# Autodesk Inventor assembly: TheLightWithinYou-ManualAttachment
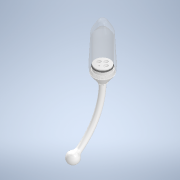
[picture p0: Inventor's stored thumbnail of the model, 180x180]
Saved by Autodesk Inventor 2021 (Build 250183000, 183)
## iProperties
Created: 2021-08-13
Part Number: TheLightWithinYou-ManualAttachment
Document SubType Name: Assembly
Designer: incep
Author: incep
## Documents named in this file (4)
- C:\Users\incep\Desktop\3D Printer Stuff\TheLightWithinYou\TheLightWithinYou-ManualAttachment.iam
- C:\Users\incep\Desktop\3D Printer Stuff\TheLightWithinYou\Bottom-V3-handle.ipt
- C:\Users\incep\Desktop\3D Printer Stuff\TheLightWithinYou\R-22-O-ring.ipt
- C:\Users\incep\Desktop\3D Printer Stuff\TheLightWithinYou\Upper-Threaded-v2.ipt
## Components (3 placed, 3 different names)
1. Bottom-V3-handle:1 — Mate:1, Flush:1, Mate:2, Mate:3
2. R-22-O-ring:1 — Mate:1, Flush:1
3. Upper-Threaded-v2:1 — Mate:2, Mate:3, Mate:4
## Relationships (5: Mate 4, Flush 1)
- Mate:1: Bottom-V3-handle:1 ↔ R-22-O-ring:1
- Flush:1: Bottom-V3-handle:1 ↔ R-22-O-ring:1
- Mate:2: Bottom-V3-handle:1 ↔ Upper-Threaded-v2:1
- Mate:3: Bottom-V3-handle:1 ↔ Upper-Threaded-v2:1
- Mate:4: Upper-Threaded-v2:1
